# Autodesk Inventor assembly: gears
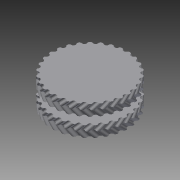
[picture p0: Inventor's stored thumbnail of the model, 180x180]
Saved by Autodesk Inventor 2013 (Build 170138000, 138)
## iProperties
Created: 2013-11-19
Part Number: gears
Document SubType Name: Assembly
Designer: employee
Author: employee
## Documents named in this file (2)
- C:\Users\employee\Desktop\GUS Simpson\_GEARS.iam
- C:\Users\employee\Desktop\GUS Simpson\_GEAR.ipt
## Components (2 placed, 1 different names)
1. _GEAR:1 — Mate:1, Mate:2, Angle:1, Mate:4
2. _GEAR:2 — Mate:1, Mate:2, Angle:1, Mate:3, Mate:5
## Relationships (6: Mate 5, Angle 1)
- Mate:1: _GEAR:1 ↔ _GEAR:2
- Mate:2 (10 mm): _GEAR:1 ↔ _GEAR:2
- Angle:1 (6 deg): _GEAR:1 ↔ _GEAR:2
- Mate:3: _GEAR:2
- Mate:4: _GEAR:1
- Mate:5 (5 mm): _GEAR:2
